# Autodesk Inventor assembly: McCrea_bodyzadokfinal_walle.ipt
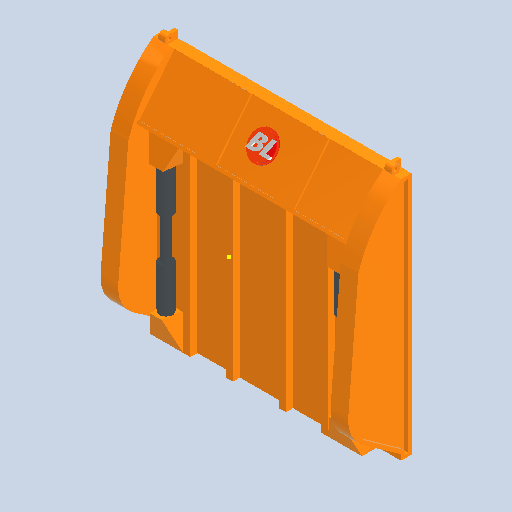
[picture p0: Inventor's stored thumbnail of the model, 512x512]
Saved by Autodesk Inventor 2022 (Build 260153000, 153)
## iProperties
Created: 2022-01-08
Part Number: McCrea_bodyzadokfinal_walle.ipt
Document SubType Name: Assembly
Designer: Lukas
Author: Lukas
## Documents named in this file (3)
- C:\Users\Lukas\Desktop\ard\3D\Walle\FINAL\lukas\McCrea_bodyzadokfinal_walle.iam
- C:\Users\Lukas\Desktop\ard\3D\Walle\FINAL\lukas\McCrea_body_zadok_walle.ipt
- C:\Users\Lukas\Desktop\ard\3D\Walle\FINAL\lukas\McCrea_bodyzadokstlp_walle.ipt
## Components (3 placed, 2 different names)
1. McCrea_body_zadok_walle:1 — Mate:1, Mate:2
2. McCrea_bodyzadokstlp_walle:1 — Mate:1
3. McCrea_bodyzadokstlp_walle:2 — Mate:2
## Relationships (2: Mate 2)
- Mate:1: McCrea_body_zadok_walle:1 ↔ McCrea_bodyzadokstlp_walle:1
- Mate:2: McCrea_body_zadok_walle:1 ↔ McCrea_bodyzadokstlp_walle:2
